# Autodesk Inventor assembly: eboard
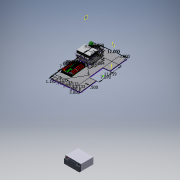
[picture p0: Inventor's stored thumbnail of the model, 180x180]
Saved by Autodesk Inventor 2016 (Build 200138000, 138)
## iProperties
Created: 2016-01-21
Part Number: eboard
Document SubType Name: Assembly
Designer: Administrator
Author: Administrator
## Documents named in this file (10)
- C:\Users\Administrator\Desktop\3192CAD\InitialRobotProto\eboard.iam
- C:\Users\Administrator\Desktop\3192CAD\InitialRobotProto\eboardbaseplate.ipt
- C:\Users\Administrator\Desktop\3192CAD\InitialRobotProto\CS_Controller_ROBORIO.ipt
- C:\Users\Administrator\Desktop\3192CAD\InitialRobotProto\CS_DistrPanel_14-806880.ipt
- C:\Users\Administrator\Desktop\3192CAD\InitialRobotProto\fc16-036_Battery.iam
- C:\Users\Administrator\Desktop\3192CAD\InitialRobotProto\ELEC_SignalLED_855PB-B12ME522.ipt
- C:\Users\Administrator\Desktop\3192CAD\InitialRobotProto\CS_WirelessBridge_DAP1522.ipt
- C:\Users\Administrator\Desktop\3192CAD\InitialRobotProto\eboardpartisland.ipt
- C:\Users\Administrator\Desktop\3192CAD\InitialRobotProto\ELEC_CircuitBreaker_CB185-120.iam
- C:\Users\Administrator\Desktop\3192CAD\InitialRobotProto\DBK_CrossHexTube_am-2241.ipt
## Components (12 placed, 9 different names)
1. eboardbaseplate:1 — Mate:1, Mate:2, Mate:9, Mate:10, Mate:11, Mate:12, Mate:17, Mate:18, Mate:19, Mate:20, Mate:21, Mate:22, Mate:23, Mate:24
2. CS_Controller_ROBORIO:1 — Mate:1, Mate:11, Mate:12
3. CS_DistrPanel_14-806880:1 — Mate:2, Mate:9, Mate:10
4. fc16-036_Battery:1 [sub-assembly]
5. ELEC_SignalLED_855PB-B12ME522:1 — Mate:13, Mate:14
6. CS_WirelessBridge_DAP1522:1 — Mate:15, Flush:3, Flush:4
7. eboardpartisland:1 — Mate:13, Mate:14, Mate:15, Mate:16, Flush:1, Flush:2, Mate:25, Mate:26, Mate:27, Flush:3, Flush:4
8. ELEC_CircuitBreaker_CB185-120:1 [sub-assembly] — Mate:16, Flush:1, Flush:2
9. DBK_CrossHexTube_am-2241:1 — Mate:17, Mate:21, Mate:26, Mate:27
10. DBK_CrossHexTube_am-2241:2 — Mate:18, Mate:22
11. DBK_CrossHexTube_am-2241:3 — Mate:20, Mate:23
12. DBK_CrossHexTube_am-2241:4 — Mate:19, Mate:24, Mate:25
## Relationships (25: Mate 21, Flush 4)
- Mate:1: eboardbaseplate:1 ↔ CS_Controller_ROBORIO:1
- Mate:2: eboardbaseplate:1 ↔ CS_DistrPanel_14-806880:1
- Mate:9: eboardbaseplate:1 ↔ CS_DistrPanel_14-806880:1
- Mate:10: eboardbaseplate:1 ↔ CS_DistrPanel_14-806880:1
- Mate:11: eboardbaseplate:1 ↔ CS_Controller_ROBORIO:1
- Mate:12: eboardbaseplate:1 ↔ CS_Controller_ROBORIO:1
- Mate:13: ELEC_SignalLED_855PB-B12ME522:1 ↔ eboardpartisland:1
- Mate:14: ELEC_SignalLED_855PB-B12ME522:1 ↔ eboardpartisland:1
- Mate:15: CS_WirelessBridge_DAP1522:1 ↔ eboardpartisland:1
- Mate:16: eboardpartisland:1 ↔ ELEC_CircuitBreaker_CB185-120:1
- Flush:1: eboardpartisland:1 ↔ ELEC_CircuitBreaker_CB185-120:1
- Flush:2 (16.5862 mm): eboardpartisland:1 ↔ ELEC_CircuitBreaker_CB185-120:1
- Mate:17: eboardbaseplate:1 ↔ DBK_CrossHexTube_am-2241:1
- Mate:18: eboardbaseplate:1 ↔ DBK_CrossHexTube_am-2241:2
- Mate:19: eboardbaseplate:1 ↔ DBK_CrossHexTube_am-2241:4
- Mate:20: eboardbaseplate:1 ↔ DBK_CrossHexTube_am-2241:3
- Mate:21: eboardbaseplate:1 ↔ DBK_CrossHexTube_am-2241:1
- Mate:22: eboardbaseplate:1 ↔ DBK_CrossHexTube_am-2241:2
- Mate:23: eboardbaseplate:1 ↔ DBK_CrossHexTube_am-2241:3
- Mate:24: eboardbaseplate:1 ↔ DBK_CrossHexTube_am-2241:4
- Mate:25: eboardpartisland:1 ↔ DBK_CrossHexTube_am-2241:4
- Mate:26: eboardpartisland:1 ↔ DBK_CrossHexTube_am-2241:1
- Mate:27: eboardpartisland:1 ↔ DBK_CrossHexTube_am-2241:1
- Flush:3 (-9.5758 mm): CS_WirelessBridge_DAP1522:1 ↔ eboardpartisland:1
- Flush:4 (13.6144 mm): CS_WirelessBridge_DAP1522:1 ↔ eboardpartisland:1
